# Autodesk Inventor assembly: doWylaniaKolek
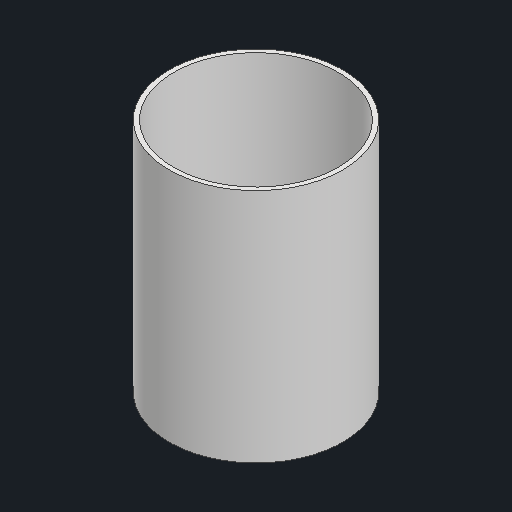
[picture p0: Inventor's stored thumbnail of the model, 512x512]
Saved by Autodesk Inventor 2023 (Build 270158000, 158)
## iProperties
Created: 2024-06-19
Part Number: doWylaniaKolek
Document SubType Name: Assembly
Designer: szymo
Author: szymo
## iProperties of the stored document pololu-universal-aluminum-mounting-hub-for-6mm-shaft-4-40-holes.ipt
Created: 2016-04-04
Part Number: pololu-universal-aluminum-mounting-hub-for-6mm-shaft-4-40-holes
Material: Generic
Description: STEP AP214
Document SubType Name: Modeling
Designer: szymo
Density: 1 g/cm^3
Appearance: Default
Sending System: SolidWorks 2016
Preprocessor: SwSTEP 2.0
Title: pololu-universal-aluminum-mounting-hub-for-6mm-shaft-4-40-holes.step
Revision Number: ANY
## Documents named in this file (5)
- D:\roboilo\robots\codename wafel - australia\3d_parts\rev4\not_in_robot_parts\formaDoWylaniaSrodek.iam
- D:\roboilo\robots\codename wafel - australia\3d_parts\rev4\not_in_robot_parts\tulejka.ipt
- **D:\roboilo\robots\codename wafel - australia\3d_parts\rev4\not_in_robot_parts\formaDoWylaniaSrodek.iam*LocalDocs*xAaaaahdaAaaaaaaaAaaaqpg0Pg*pololu-universal-aluminum-mounting-hub-for-6mm-shaft-4-40-holes.ipt
- **D:\roboilo\robots\codename wafel - australia\3d_parts\rev4\not_in_robot_parts\doWylaniaKolek.iam*LocalDocs*xAaaaahdaAaaaaaaaAaaaqpg0Pg*pololu-universal-aluminum-mounting-hub-for-6mm-shaft-4-40-holes.ipt
- D:\roboilo\robots\codename wafel - australia\3d_parts\rev4\not_in_robot_parts\pololu-universal-aluminum-mounting-hub-for-6mm-shaft-4-40-holes.step
## Components (2 placed, 2 different names)
1. pololu-universal-aluminum-mounting-hub-for-6mm-shaft-4-40-holes:1 — Mate:1, Flush:1
2. tulejka:1 — Mate:1, Flush:1
## Relationships (2: Mate 1, Flush 1)
- Mate:1: pololu-universal-aluminum-mounting-hub-for-6mm-shaft-4-40-holes:1 ↔ tulejka:1
- Flush:1: pololu-universal-aluminum-mounting-hub-for-6mm-shaft-4-40-holes:1 ↔ tulejka:1
